# Autodesk Inventor assembly: ASY ANP 1424 FDS way 4
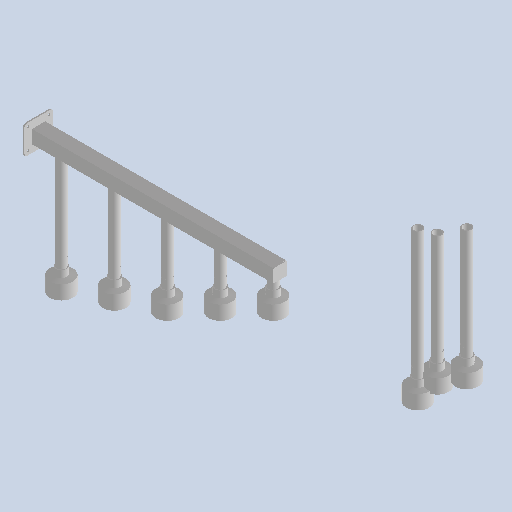
[picture p0: Inventor's stored thumbnail of the model, 512x512]
Saved by Autodesk Inventor 2025 (Build 290162010, 162A)
## iProperties
Created: 2025-07-02
Part Number: ASY ANP 1424 FDS way 4
Document SubType Name: Assembly
Designer: admin
Author: user
## Documents named in this file (12)
- C:\Users\pokla\Documents\Inventor\ANP--Antipayuta\FDS 1400\ASY ANP 1424 FDS way 4.iam
- C:\Users\pokla\Documents\Inventor\ANP--Antipayuta\FDS 1400\ANP 1434 FDS WAY tube4.ipt
- C:\Users\pokla\Documents\Inventor\ANP--Antipayuta\FDS 1400\ANP 1425 FDS Way FLANGE.ipt
- C:\Users\pokla\Documents\Inventor\ANP--Antipayuta\FDS 1400\ANP 1426 FDS way cup.ipt
- C:\Users\pokla\Documents\Inventor\ANP--Antipayuta\FDS 1400\ANP dummy filter element.ipt
- C:\Users\pokla\Documents\Inventor\ANP--Antipayuta\FDS 1400\ANP dummy pipe nippel.ipt
- C:\Users\pokla\Documents\Inventor\ANP--Antipayuta\FDS 1400\ANP 1445 FDS thread  tube5.ipt
- C:\Users\pokla\Documents\Inventor\ANP--Antipayuta\FDS 1400\ANP 1446 FDS thread  tube6.ipt
- C:\Users\pokla\Documents\Inventor\ANP--Antipayuta\FDS 1400\ANP 1447 FDS thread  tube7.ipt
- C:\Users\pokla\Documents\Inventor\ANP--Antipayuta\FDS 1400\ANP 1448 FDS thread  tube8.ipt
- C:\Users\pokla\Documents\Inventor\ANP--Antipayuta\FDS 1400\ANP 1449 FDS thread  tube9.ipt
- C:\Users\pokla\Documents\Inventor\ANP--Antipayuta\FDS 1400\ANP 1451 FDS thread  tube10.ipt
## Components (26 placed, 11 different names)
1. ANP 1434 FDS WAY tube4.ipt:1 — Rigid:34, Rigid:35, Rigid:36, Rigid:50, Rigid:51, Rigid:52, Rigid:53, Rigid:54, Rigid:55, Rigid:39
2. ANP 1425 FDS Way FLANGE.ipt:1 — Rigid:34
3. ANP 1426 FDS way cup.ipt:1 — Rigid:35
4. ANP dummy filter element.ipt:1 — Rigid:1
5. ANP dummy pipe nippel.ipt:1 — Rigid:1, Rigid:44
6. ANP dummy filter element.ipt:2 — Rigid:6
7. ANP dummy pipe nippel.ipt:2 — Rigid:6, Rigid:46
8. ANP dummy filter element.ipt:3 — Rigid:11
9. ANP dummy pipe nippel.ipt:3 — Rigid:11, Rigid:47
10. ANP dummy filter element.ipt:4 — Rigid:14
11. ANP dummy pipe nippel.ipt:4 — Rigid:14, Rigid:45
12. ANP dummy filter element.ipt:5 — Rigid:26
13. ANP dummy pipe nippel.ipt:5 — Rigid:26, Rigid:49
14. ANP dummy filter element.ipt:6 — Rigid:27
15. ANP dummy pipe nippel.ipt:6 — Rigid:27, Rigid:48
16. ANP dummy filter element.ipt:7 — Rigid:33
17. ANP dummy pipe nippel.ipt:7 — Rigid:36, Rigid:33
18. ANP 1445 FDS thread  tube5.ipt:1 — Rigid:50, Rigid:49
19. ANP 1446 FDS thread  tube6.ipt:1 — Rigid:51, Rigid:48
20. ANP 1447 FDS thread  tube7.ipt:1 — Rigid:52, Rigid:47
21. ANP 1448 FDS thread  tube8.ipt:1 — Rigid:53, Rigid:46
22. ANP 1449 FDS thread  tube9.ipt:1 — Rigid:54, Rigid:45
23. ANP 1451 FDS thread  tube10.ipt:1 — Rigid:55, Rigid:44
24. ANP dummy filter element.ipt:9
25. ANP dummy pipe nippel.ipt:9
26. ANP 1446 FDS thread  tube6.ipt:2 — Rigid:39
## Relationships (25: WeldJoint 25)
- Rigid:1 [WeldJoint]: ANP dummy filter element.ipt:1 ↔ ANP dummy pipe nippel.ipt:1
- Rigid:6 [WeldJoint]: ANP dummy filter element.ipt:2 ↔ ANP dummy pipe nippel.ipt:2
- Rigid:34 [WeldJoint] (2 mm): ANP 1434 FDS WAY tube4.ipt:1 ↔ ANP 1425 FDS Way FLANGE.ipt:1
- Rigid:35 [WeldJoint]: ANP 1434 FDS WAY tube4.ipt:1 ↔ ANP 1426 FDS way cup.ipt:1
- Rigid:11 [WeldJoint]: ANP dummy filter element.ipt:3 ↔ ANP dummy pipe nippel.ipt:3
- Rigid:14 [WeldJoint]: ANP dummy filter element.ipt:4 ↔ ANP dummy pipe nippel.ipt:4
- Rigid:26 [WeldJoint]: ANP dummy filter element.ipt:5 ↔ ANP dummy pipe nippel.ipt:5
- Rigid:27 [WeldJoint]: ANP dummy filter element.ipt:6 ↔ ANP dummy pipe nippel.ipt:6
- Rigid:36 [WeldJoint]: ANP 1434 FDS WAY tube4.ipt:1 ↔ ANP dummy pipe nippel.ipt:7
- Rigid:33 [WeldJoint]: ANP dummy filter element.ipt:7 ↔ ANP dummy pipe nippel.ipt:7
- Rigid:50 [WeldJoint]: ANP 1434 FDS WAY tube4.ipt:1 ↔ ANP 1445 FDS thread  tube5.ipt:1
- Rigid:49 [WeldJoint]: ANP dummy pipe nippel.ipt:5 ↔ ANP 1445 FDS thread  tube5.ipt:1
- Rigid:51 [WeldJoint]: ANP 1434 FDS WAY tube4.ipt:1 ↔ ANP 1446 FDS thread  tube6.ipt:1
- Rigid:48 [WeldJoint]: ANP dummy pipe nippel.ipt:6 ↔ ANP 1446 FDS thread  tube6.ipt:1
- Rigid:52 [WeldJoint]: ANP 1434 FDS WAY tube4.ipt:1 ↔ ANP 1447 FDS thread  tube7.ipt:1
- Rigid:47 [WeldJoint]: ANP dummy pipe nippel.ipt:3 ↔ ANP 1447 FDS thread  tube7.ipt:1
- Rigid:53 [WeldJoint]: ANP 1434 FDS WAY tube4.ipt:1 ↔ ANP 1448 FDS thread  tube8.ipt:1
- Rigid:46 [WeldJoint]: ANP dummy pipe nippel.ipt:2 ↔ ANP 1448 FDS thread  tube8.ipt:1
- Rigid:54 [WeldJoint]: ANP 1434 FDS WAY tube4.ipt:1 ↔ ANP 1449 FDS thread  tube9.ipt:1
- Rigid:45 [WeldJoint]: ANP dummy pipe nippel.ipt:4 ↔ ANP 1449 FDS thread  tube9.ipt:1
- Rigid:55 [WeldJoint]: ANP 1434 FDS WAY tube4.ipt:1 ↔ ANP 1451 FDS thread  tube10.ipt:1
- Rigid:44 [WeldJoint]: ANP dummy pipe nippel.ipt:1 ↔ ANP 1451 FDS thread  tube10.ipt:1
- [WeldJoint]: ANP dummy filter element.ipt:9 ↔ ANP dummy pipe nippel.ipt:9
- [WeldJoint]: ANP dummy pipe nippel.ipt:9 ↔ ANP 1446 FDS thread  tube6.ipt:2
- Rigid:39 [WeldJoint]: ANP 1434 FDS WAY tube4.ipt:1 ↔ ANP 1446 FDS thread  tube6.ipt:2
## Named parameters: d36_d25 = 0 mm, d37_d13 = 0 mm
